# Autodesk Inventor assembly: Mounted Camera w Lens
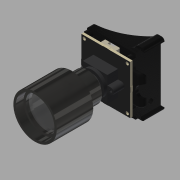
[picture p0: Inventor's stored thumbnail of the model, 180x180]
Saved by Autodesk Inventor 2020 (Build 240168000, 168)
## iProperties
Created: 2019-05-09
Part Number: Mounted Camera w Lens
Document SubType Name: Assembly
Designer: Ben
Author: Ben
## Documents named in this file (4)
- C:\Users\Ben\Documents\Inventor\HydraVivarium\Mounted Camera w Lens.iam
- C:\Users\Ben\Documents\Inventor\HydraVivarium\Camera Mount 01.ipt
- C:\Users\Ben\Documents\Inventor\HydraVivarium\M12 2.8-12mm F1.4 Lens.ipt
- C:\Users\Ben\Documents\Inventor\HydraVivarium\Spinel USB Camera 01 trimmed.ipt
## Components (3 placed, 3 different names)
1. Camera Mount 01:1 — Flush:1, Mate:1, Mate:2, Mate:3
2. Spinel USB Camera 01 trimmed:1 — Flush:1, Mate:1, Mate:2
3. M12 2.8-12mm F1.4 Lens:1 — Mate:3
## Relationships (4: Mate 3, Flush 1)
- Flush:1: Camera Mount 01:1 ↔ Spinel USB Camera 01 trimmed:1
- Mate:1: Camera Mount 01:1 ↔ Spinel USB Camera 01 trimmed:1
- Mate:2: Camera Mount 01:1 ↔ Spinel USB Camera 01 trimmed:1
- Mate:3: Camera Mount 01:1 ↔ M12 2.8-12mm F1.4 Lens:1
